# Autodesk Inventor assembly: FlyWheelAssembly
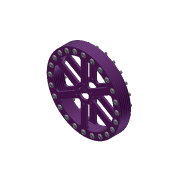
[picture p0: Inventor's stored thumbnail of the model, 180x180]
Saved by Autodesk Inventor 2012 (Build 160160000, 160)
## iProperties
Created: 2012-01-20
Part Number: FlyWheelAssembly
Document SubType Name: Assembly
Designer: JesseK
Mass: 1243.13 g
Surface Area: 2322.21 cm^2
Volume: 393.552 cm^3
Density: 3.15873 g/cm^3
Author: JesseK
## Documents named in this file (4)
- Z:\UserData\Documents\Inventor\team1885frc\Robot2012\Shooter\FlyWheelAssembly.iam
- Z:\UserData\Documents\Inventor\team1885frc\Robot2012\Shooter\FlyWheelBase.ipt
- Z:\UserData\Documents\Inventor\team1885frc\Robot2012\Shooter\FlyWheelWeight.ipt
- Z:\UserData\Documents\Inventor\team1885frc\Robot2012\Shooter\ShooterWeight.ipt
## Components (30 placed, 3 different names)
1. FlyWheelBase:1 — Mate:1, Mate:3, Mate:10, Mate:11, Mate:12, Mate:13, Mate:14, Mate:15, Mate:16, Mate:17, Mate:18, Mate:19, Mate:20, Mate:21, Mate:22, Mate:23, Mate:24, Mate:25, Mate:26, Mate:27, Mate:28, Mate:29, Mate:30, Mate:31, Mate:32, Mate:33, Mate:34, Mate:35, Mate:36, Mate:37, Mate:38, Mate:39, Mate:40, Mate:41, Mate:42, Mate:43, Mate:44, Mate:45, Mate:46, Mate:47, Mate:48, Mate:49, Mate:50, Mate:51, Mate:52, Mate:53, Mate:54, Mate:55, Mate:56, Mate:57
2. FlyWheelBase:2 — Mate:7
3. FlyWheelWeight:1 — Mate:1, Mate:2, Mate:3, Mate:4
4. FlyWheelWeight:2 — Mate:2, Mate:4, Mate:5, Mate:8
5. FlyWheelWeight:3 — Mate:6, Mate:7, Mate:9
6. FlyWheelWeight:4 — Mate:5, Mate:6, Mate:8, Mate:9
7. ShooterWeight:1 — Mate:10, Mate:52
8. ShooterWeight:2 — Mate:11, Mate:57
9. ShooterWeight:3 — Mate:12, Mate:51
10. ShooterWeight:4 — Mate:13, Mate:50
11. ShooterWeight:5 — Mate:14, Mate:49
12. ShooterWeight:6 — Mate:15, Mate:48
13. ShooterWeight:7 — Mate:16, Mate:47
14. ShooterWeight:8 — Mate:17, Mate:46
15. ShooterWeight:9 — Mate:18, Mate:45
16. ShooterWeight:10 — Mate:19, Mate:44
17. ShooterWeight:11 — Mate:20, Mate:43
18. ShooterWeight:12 — Mate:21, Mate:42
19. ShooterWeight:13 — Mate:22, Mate:41
20. ShooterWeight:14 — Mate:23, Mate:40
21. ShooterWeight:15 — Mate:24, Mate:39
22. ShooterWeight:16 — Mate:25, Mate:38
23. ShooterWeight:17 — Mate:26, Mate:37
24. ShooterWeight:18 — Mate:27, Mate:36
25. ShooterWeight:19 — Mate:30, Mate:54
26. ShooterWeight:20 — Mate:32, Mate:34
27. ShooterWeight:21 — Mate:33, Mate:35
28. ShooterWeight:22 — Mate:31, Mate:53
29. ShooterWeight:23 — Mate:29, Mate:55
30. ShooterWeight:24 — Mate:28, Mate:56
## Relationships (57: Mate 57)
- Mate:1: FlyWheelBase:1 ↔ FlyWheelWeight:1
- Mate:2: FlyWheelWeight:1 ↔ FlyWheelWeight:2
- Mate:3: FlyWheelBase:1 ↔ FlyWheelWeight:1
- Mate:4: FlyWheelWeight:1 ↔ FlyWheelWeight:2
- Mate:5: FlyWheelWeight:2 ↔ FlyWheelWeight:4
- Mate:6: FlyWheelWeight:3 ↔ FlyWheelWeight:4
- Mate:7: FlyWheelBase:2 ↔ FlyWheelWeight:3
- Mate:8: FlyWheelWeight:2 ↔ FlyWheelWeight:4
- Mate:9: FlyWheelWeight:3 ↔ FlyWheelWeight:4
- Mate:10: FlyWheelBase:1 ↔ ShooterWeight:1
- Mate:11: FlyWheelBase:1 ↔ ShooterWeight:2
- Mate:12: FlyWheelBase:1 ↔ ShooterWeight:3
- Mate:13: FlyWheelBase:1 ↔ ShooterWeight:4
- Mate:14: FlyWheelBase:1 ↔ ShooterWeight:5
- Mate:15: FlyWheelBase:1 ↔ ShooterWeight:6
- Mate:16: FlyWheelBase:1 ↔ ShooterWeight:7
- Mate:17: FlyWheelBase:1 ↔ ShooterWeight:8
- Mate:18: FlyWheelBase:1 ↔ ShooterWeight:9
- Mate:19: FlyWheelBase:1 ↔ ShooterWeight:10
- Mate:20: FlyWheelBase:1 ↔ ShooterWeight:11
- Mate:21: FlyWheelBase:1 ↔ ShooterWeight:12
- Mate:22: FlyWheelBase:1 ↔ ShooterWeight:13
- Mate:23: FlyWheelBase:1 ↔ ShooterWeight:14
- Mate:24: FlyWheelBase:1 ↔ ShooterWeight:15
- Mate:25: FlyWheelBase:1 ↔ ShooterWeight:16
- Mate:26: FlyWheelBase:1 ↔ ShooterWeight:17
- Mate:27: FlyWheelBase:1 ↔ ShooterWeight:18
- Mate:28: FlyWheelBase:1 ↔ ShooterWeight:24
- Mate:29: FlyWheelBase:1 ↔ ShooterWeight:23
- Mate:30: FlyWheelBase:1 ↔ ShooterWeight:19
- Mate:31: FlyWheelBase:1 ↔ ShooterWeight:22
- Mate:32: FlyWheelBase:1 ↔ ShooterWeight:20
- Mate:33: FlyWheelBase:1 ↔ ShooterWeight:21
- Mate:34: FlyWheelBase:1 ↔ ShooterWeight:20
- Mate:35: FlyWheelBase:1 ↔ ShooterWeight:21
- Mate:36: FlyWheelBase:1 ↔ ShooterWeight:18
- Mate:37: FlyWheelBase:1 ↔ ShooterWeight:17
- Mate:38: FlyWheelBase:1 ↔ ShooterWeight:16
- Mate:39: FlyWheelBase:1 ↔ ShooterWeight:15
- Mate:40: FlyWheelBase:1 ↔ ShooterWeight:14
- Mate:41: FlyWheelBase:1 ↔ ShooterWeight:13
- Mate:42: FlyWheelBase:1 ↔ ShooterWeight:12
- Mate:43: FlyWheelBase:1 ↔ ShooterWeight:11
- Mate:44: FlyWheelBase:1 ↔ ShooterWeight:10
- Mate:45: FlyWheelBase:1 ↔ ShooterWeight:9
- Mate:46: FlyWheelBase:1 ↔ ShooterWeight:8
- Mate:47: FlyWheelBase:1 ↔ ShooterWeight:7
- Mate:48: FlyWheelBase:1 ↔ ShooterWeight:6
- Mate:49: FlyWheelBase:1 ↔ ShooterWeight:5
- Mate:50: FlyWheelBase:1 ↔ ShooterWeight:4
- Mate:51: FlyWheelBase:1 ↔ ShooterWeight:3
- Mate:52: FlyWheelBase:1 ↔ ShooterWeight:1
- Mate:53: FlyWheelBase:1 ↔ ShooterWeight:22
- Mate:54: FlyWheelBase:1 ↔ ShooterWeight:19
- Mate:55: FlyWheelBase:1 ↔ ShooterWeight:23
- Mate:56: FlyWheelBase:1 ↔ ShooterWeight:24
- Mate:57: FlyWheelBase:1 ↔ ShooterWeight:2
